# Autodesk Inventor assembly: Shaft Collar Set Screw_MIR1
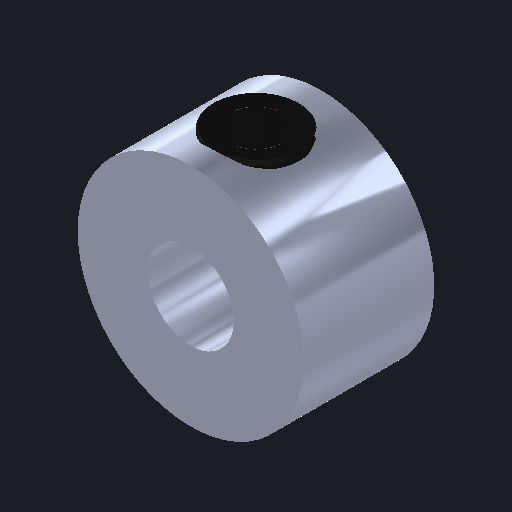
[picture p0: Inventor's stored thumbnail of the model, 512x512]
Saved by Autodesk Inventor 2024 (Build 280153000, 153)
## iProperties
Created: 2022-08-01
Part Number: Shaft Collar Set Screw_MIR1
Document SubType Name: Assembly
Designer: macbook
Author: ylu12
## Documents named in this file (3)
- \\Mac\Home\Desktop\code\7899V-VRC-OVER-UNDER\Cad\VEX-CAD-Inventor-1.4.0\Motion\Shaft LS\Shaft Collar Metal\Shaft Collar Set Screw_MIR1.iam
- \\Mac\Home\Desktop\code\7899V-VRC-OVER-UNDER\Cad\VEX-CAD-Inventor-1.4.0\Motion\Reference Files\Shaft Collar Metal_MIR2.ipt
- \\Mac\Home\Desktop\code\7899V-VRC-OVER-UNDER\Cad\VEX-CAD-Inventor-1.4.0\Motion\Reference Files\Set Screw_MIR1.ipt
## Components (2 placed, 2 different names)
1. Shaft Collar Metal_MIR2:1 — Flush:1, Mate:2, Mate:1, Insert:1
2. Set Screw_MIR1:1 — Insert:1
## Relationships (4: Mate 2, Flush 1, Insert 1)
- Flush:1: Shaft Collar Metal_MIR2:1
- Mate:2: Shaft Collar Metal_MIR2:1
- Mate:1: Shaft Collar Metal_MIR2:1
- Insert:1: Shaft Collar Metal_MIR2:1 ↔ Set Screw_MIR1:1
